# Autodesk Inventor assembly: OneWheelBlock
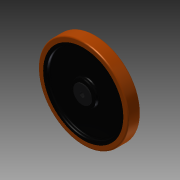
[picture p0: Inventor's stored thumbnail of the model, 180x180]
Saved by Autodesk Inventor 2014 SP1 (Build 180222100, 222)
## iProperties
Created: 2015-04-11
Part Number: OneWheelBlock
Document SubType Name: Assembly
Designer: david
Mass: 27.8756 g
Surface Area: 169.195 cm^2
Volume: 26.891 cm^3
Density: 1.03661 g/cm^3
Author: david
## Documents named in this file (4)
- C:\Users\asus\Documents\Autodesk\Projects\AUSBEEDone\Components\BaneBots\OneWheelBlock.iam
- C:\Users\asus\Documents\Autodesk\Projects\AUSBEEDone\Components\BaneBots\Hub_Hex_4mmBore_1Wide.ipt
- C:\Users\asus\Documents\Autodesk\Projects\AUSBEEDone\Components\BaneBots\Wheel_73mm-10mm-HexMount_40A.ipt
- C:\Users\asus\Documents\Autodesk\Projects\AUSBEEDone\Components\BaneBots\SetScrew.ipt
## Components (3 placed, 3 different names)
1. Hub_Hex_4mmBore_1Wide:1 — Mate:1, Mate:2, Mate:3, Mate:4
2. Wheel_73mm-10mm-HexMount_40A:1 — Mate:1, Mate:2, Mate:3
3. SetScrew:1 — Mate:4
## Relationships (4: Mate 4)
- Mate:1: Hub_Hex_4mmBore_1Wide:1 ↔ Wheel_73mm-10mm-HexMount_40A:1
- Mate:2: Hub_Hex_4mmBore_1Wide:1 ↔ Wheel_73mm-10mm-HexMount_40A:1
- Mate:3: Hub_Hex_4mmBore_1Wide:1 ↔ Wheel_73mm-10mm-HexMount_40A:1
- Mate:4: Hub_Hex_4mmBore_1Wide:1 ↔ SetScrew:1
